# Autodesk Inventor assembly: Ethernet
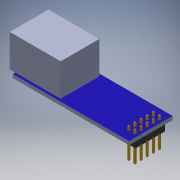
[picture p0: Inventor's stored thumbnail of the model, 180x180]
Saved by Autodesk Inventor 2018 (Build 220112000, 112)
## iProperties
Created: 2017-04-09
Part Number: Ethernet
Document SubType Name: Assembly
Designer: dkt01
Author: dkt01
## Documents named in this file (3)
- C:\Users\dktur\Dropbox\StackLightMonitor\CAD\Ethernet.iam
- C:\Users\dktur\Dropbox\StackLightMonitor\CAD\Ethernet.ipt
- C:\Users\dktur\Dropbox\StackLightMonitor\CAD\MaleHeader-02.iam
## Components (2 placed, 2 different names)
1. Ethernet:1 — Mate:1, Tangent:1, Tangent:2, Tangent:3
2. MaleHeader-02:1 [sub-assembly] — Mate:1, Tangent:1, Tangent:2, Tangent:3
## Relationships (4: Tangent 3, Mate 1)
- Mate:1: Ethernet:1 ↔ MaleHeader-02:1
- Tangent:1: Ethernet:1 ↔ MaleHeader-02:1
- Tangent:2: Ethernet:1 ↔ MaleHeader-02:1
- Tangent:3: Ethernet:1 ↔ MaleHeader-02:1
